# Autodesk Inventor assembly: Ensamblaje_Carcaza_sup_ch
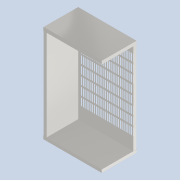
[picture p0: Inventor's stored thumbnail of the model, 180x180]
Saved by Autodesk Inventor 2021 (Build 250183000, 183)
## iProperties
Created: 2021-05-16
Part Number: Ensamblaje_Carcaza_sup_ch
Document SubType Name: Assembly
Designer: Admin
Mass: 2946.62 g
Surface Area: 11445.5 cm^2
Volume: 374.317 cm^3
Density: 7.872 g/cm^3
Author: Admin
## Documents named in this file (4)
- E:\Documentos\Documentos\Michael_Rodriguez\Universidad_Nacional\Doceaba matricula\PAI\Proyecto PAI\Proyecto_PAI_2021\01 CAD\Ensamblaje_Carcaza_sup_ch.iam
- E:\Documentos\Documentos\Michael_Rodriguez\Universidad_Nacional\Doceaba matricula\PAI\Proyecto PAI\Proyecto_PAI_2021\01 CAD\Tapa_superior_sup_ch.ipt
- E:\Documentos\Documentos\Michael_Rodriguez\Universidad_Nacional\Doceaba matricula\PAI\Proyecto PAI\Proyecto_PAI_2021\01 CAD\Tapa_superior_izq_ch.ipt
- E:\Documentos\Documentos\Michael_Rodriguez\Universidad_Nacional\Doceaba matricula\PAI\Proyecto PAI\Proyecto_PAI_2021\01 CAD\Tapa_superior_der_ch.ipt
## Components (3 placed, 3 different names)
1. Tapa_superior_sup_ch:1 — Coincidencia:1, Coincidencia:2, Coincidencia:3, Coincidencia:4, Coincidencia:5, Coincidencia:6
2. Tapa_superior_izq_ch:1 — Coincidencia:4, Coincidencia:5, Coincidencia:6
3. Tapa_superior_der_ch:1 — Coincidencia:1, Coincidencia:2, Coincidencia:3
## Relationships (6: Mate 6)
- Coincidencia:1 [Mate]: Tapa_superior_sup_ch:1 ↔ Tapa_superior_der_ch:1
- Coincidencia:2 [Mate]: Tapa_superior_sup_ch:1 ↔ Tapa_superior_der_ch:1
- Coincidencia:3 [Mate]: Tapa_superior_sup_ch:1 ↔ Tapa_superior_der_ch:1
- Coincidencia:4 [Mate]: Tapa_superior_sup_ch:1 ↔ Tapa_superior_izq_ch:1
- Coincidencia:5 [Mate]: Tapa_superior_sup_ch:1 ↔ Tapa_superior_izq_ch:1
- Coincidencia:6 [Mate]: Tapa_superior_sup_ch:1 ↔ Tapa_superior_izq_ch:1
